# Autodesk Inventor assembly: Big Shaft Motor Assembly
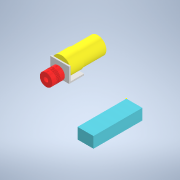
[picture p0: Inventor's stored thumbnail of the model, 180x180]
Saved by Autodesk Inventor 2022 (Build 260153000, 153)
## iProperties
Created: 2021-06-03
Part Number: Big Shaft Motor Assembly
Document SubType Name: Assembly
Designer: jrcol
Author: jrcol
## Documents named in this file (5)
- C:\Users\jrcol\Desktop\Solar-Lab-Files\Smart Drill\Big Shaft Motor Assembly.iam
- C:\Users\jrcol\Desktop\Solar-Lab-Files\Smart Drill\Big Motor.ipt
- C:\Users\jrcol\Desktop\Solar-Lab-Files\Smart Drill\Big shaft coupling.ipt
- C:\Users\jrcol\Desktop\Solar-Lab-Files\Smart Drill\Big Motor Bracket.ipt
- C:\Users\jrcol\Desktop\Solar-Lab-Files\Smart Drill\Battery.ipt
## Components (4 placed, 4 different names)
1. Big Motor:1 — Mate:1
2. Big shaft coupling:1
3. Big Motor Bracket:1 — Mate:1
4. Battery:1
## Relationships (1: Mate 1)
- Mate:1: Big Motor:1 ↔ Big Motor Bracket:1
